# Autodesk Inventor assembly: Baseplate Assembley
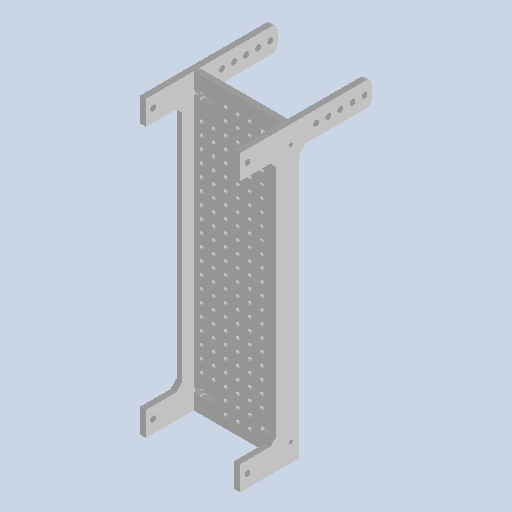
[picture p0: Inventor's stored thumbnail of the model, 512x512]
Saved by Autodesk Inventor 2024.1 (Build 281209000, 209)
## iProperties
Created: 2022-07-07
Part Number: Baseplate Assembley
Document SubType Name: Assembly
Designer: abdoo
Author: abdoo
## Documents named in this file (3)
- C:\Users\udayk\OneDrive\Desktop\Year 1\Engineer IP13\Project 3\Thurs-08 Modelling\2. Hopper Assembly\2. Hopper Assembly\Baseplate Assembley.iam
- C:\Users\udayk\OneDrive\Desktop\Year 1\Engineer IP13\Project 3\Thurs-08 Modelling\2. Hopper Assembly\2. Hopper Assembly\Mounting Wall.ipt
- C:\Users\udayk\OneDrive\Desktop\Year 1\Engineer IP13\Project 3\Thurs-08 Modelling\2. Hopper Assembly\2. Hopper Assembly\Mounting Plate.ipt
## Components (3 placed, 2 different names)
1. Mounting Wall:1 — Mate:3, Mate:4, Flush:2
2. Mounting Wall:2 — Mate:1, Mate:2, Flush:1
3. Mounting Plate:1 — Mate:1, Mate:2, Flush:1, Mate:3, Mate:4, Flush:2
## Relationships (6: Mate 4, Flush 2)
- Mate:1: Mounting Wall:2 ↔ Mounting Plate:1
- Mate:2: Mounting Wall:2 ↔ Mounting Plate:1
- Flush:1: Mounting Wall:2 ↔ Mounting Plate:1
- Mate:3: Mounting Wall:1 ↔ Mounting Plate:1
- Mate:4: Mounting Wall:1 ↔ Mounting Plate:1
- Flush:2: Mounting Wall:1 ↔ Mounting Plate:1
